# Autodesk Inventor assembly: Subensamble_mesa
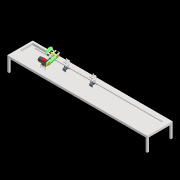
[picture p0: Inventor's stored thumbnail of the model, 180x180]
Saved by Autodesk Inventor 2021 (Build 250183000, 183)
## iProperties
Created: 2021-04-29
Part Number: Subensamble_mesa
Document SubType Name: Assembly
Designer: Admin
Author: Admin
## Documents named in this file (18)
- C:\Users\maaro\Documents\UNAL\Automatización de Procesos de Manufactura\Github\Proyecto_APM\CADs estaciones a automatizar\Estación corte\Subensamble_mesa.iam
- C:\Users\maaro\Documents\UNAL\Automatización de Procesos de Manufactura\Github\Proyecto_APM\CADs estaciones a automatizar\Estación corte\Mesa_cortadora.ipt
- C:\Users\maaro\Documents\UNAL\Automatización de Procesos de Manufactura\Github\Proyecto_APM\CADs estaciones a automatizar\Estación corte\Pata_mesa.ipt
- C:\Users\maaro\Documents\UNAL\Automatización de Procesos de Manufactura\Github\Proyecto_APM\CADs estaciones a automatizar\Estación corte\Subensamble_cortadora.iam
- C:\Users\maaro\Documents\UNAL\Automatización de Procesos de Manufactura\Github\Proyecto_APM\CADs estaciones a automatizar\Estación corte\Tubo-2_1_8.ipt
- C:\Users\maaro\Documents\UNAL\Automatización de Procesos de Manufactura\Github\Proyecto_APM\CADs estaciones a automatizar\Estación corte\Base soporte tubos.ipt
- C:\Users\maaro\Documents\UNAL\Automatización de Procesos de Manufactura\Github\Proyecto_APM\CADs estaciones a automatizar\Estación corte\193992 DSNU-32-60-PPS-A---(60PPSA---00--0-------0).iam
- C:\Users\maaro\Documents\UNAL\Automatización de Procesos de Manufactura\Github\Proyecto_APM\CADs estaciones a automatizar\Estación corte\Eje roscado base soporte tubo.ipt
- C:\Users\maaro\Documents\UNAL\Automatización de Procesos de Manufactura\Github\Proyecto_APM\CADs estaciones a automatizar\Estación corte\Soporte Superior Tubos.ipt
- C:\Users\maaro\Documents\UNAL\Automatización de Procesos de Manufactura\Github\Proyecto_APM\CADs estaciones a automatizar\Estación corte\Soporte Pistón.ipt
- C:\Users\maaro\Documents\Inventor\Content Center Files\R2021\en-US\ISO 4035(2)\ISO 4035 - M16 - ISO.ipt
- C:\Users\maaro\Documents\UNAL\Automatización de Procesos de Manufactura\Github\Proyecto_APM\CADs estaciones a automatizar\Estación corte\Eje roscado base soporte tubo_MIR.ipt
- C:\Users\maaro\Documents\UNAL\Automatización de Procesos de Manufactura\Github\Proyecto_APM\CADs estaciones a automatizar\Estación corte\193992 DSNU-32-60-PPS-A---(60PPSA---00--0-------0)_MIR.iam
- C:\Users\maaro\Documents\UNAL\Automatización de Procesos de Manufactura\Github\Proyecto_APM\CADs estaciones a automatizar\Estación corte\Base soporte tubos_MIR.ipt
- C:\Users\maaro\Documents\UNAL\Automatización de Procesos de Manufactura\Github\Proyecto_APM\CADs estaciones a automatizar\Estación corte\Eje roscado base soporte tubo_MIR1.ipt
- C:\Users\maaro\Documents\UNAL\Automatización de Procesos de Manufactura\Github\Proyecto_APM\CADs estaciones a automatizar\Estación corte\Soporte Superior Tubos_MIR.ipt
- C:\Users\maaro\Documents\UNAL\Automatización de Procesos de Manufactura\Github\Proyecto_APM\CADs estaciones a automatizar\Estación corte\Soporte Pistón_MIR.ipt
- C:\Users\maaro\Documents\UNAL\Automatización de Procesos de Manufactura\Github\Proyecto_APM\CADs estaciones a automatizar\Estación corte\Eje roscado base soporte tubo_MIR_MIR.ipt
## Components (36 placed, 17 different names)
1. Mesa_cortadora:1 — Coincidencia:1, Coincidencia:2, Coincidencia:3, Coincidencia:4, Coincidencia:5, Coincidencia:6, Coincidencia:7, Coincidencia:8, Coincidencia:9, Coincidencia:10, Coincidencia:11, Coincidencia:12, Coincidencia:13, Coincidencia:14, Mate:15, Flush:1, Flush:2, Mate:16, Flush:3, Mate:80, Flush:17
2. Pata_mesa:1 — Coincidencia:7, Coincidencia:8, Coincidencia:9
3. Pata_mesa:2 — Coincidencia:1, Coincidencia:2, Coincidencia:3
4. Pata_mesa:3 — Coincidencia:4, Coincidencia:5, Coincidencia:6
5. Pata_mesa:4 — Coincidencia:10, Coincidencia:11, Coincidencia:12
6. Subensamble_cortadora:1 [sub-assembly] — Coincidencia:13, Coincidencia:14
7. Tubo-2_1_8:1 — Tangent:1, Tangent:2, Flush:7
8. Base soporte tubos:1 — Mate:15, Tangent:1, Tangent:2, Flush:1, Flush:2
9. 193992 DSNU-32-60-PPS-A---(60PPSA---00--0-------0):2 [sub-assembly] — Mate:18, Flush:10, Flush:11
10. Base soporte tubos:2 — Mate:16, Flush:3, Flush:5, Flush:6, Flush:8, Flush:9, Mate:23, Mate:25, Mate:31, Mate:36, Mate:37, Mate:38, Flush:12
11. Eje roscado base soporte tubo:1 — Flush:5, Flush:6, Mate:20, Mate:22, Mate:24, Mate:26, Mate:31, Mate:32, Mate:33
12. Soporte Superior Tubos:1 — Flush:7, Flush:8, Flush:9, Mate:18, Symmetry:1, Mate:33
13. Soporte Pistón:1 — Flush:10, Flush:11, Mate:19, Mate:21, Symmetry:1, Mate:32, Mate:34, Mate:35, Flush:13, Mate:39
14. ISO 4035 M16:1 — Mate:21, Mate:22
15. ISO 4035 M16:2 — Mate:19, Mate:20
16. ISO 4035 M16:3 — Mate:23, Mate:24
17. ISO 4035 M16:4 — Mate:25, Mate:26
18. Eje roscado base soporte tubo_MIR:1 — Mate:27, Mate:28, Mate:29, Mate:30, Mate:38, Flush:12, Flush:13, Mate:39
19. ISO 4035 M16:5 — Mate:27, Mate:34
20. ISO 4035 M16:6 — Mate:28, Mate:35
21. ISO 4035 M16:7 — Mate:29, Mate:37
22. ISO 4035 M16:8 — Mate:30, Mate:36
23. 193992 DSNU-32-60-PPS-A---(60PPSA---00--0-------0)_MIR:1 [sub-assembly] — Mate:44, Mate:48, Mate:49
24. Base soporte tubos_MIR:1 — Mate:40, Mate:41, Mate:42, Mate:45, Mate:46, Mate:55, Mate:57, Flush:16, Mate:59, Mate:64, Mate:66, Mate:72, Mate:74, Mate:76, Mate:78, Mate:80, Flush:17
25. Eje roscado base soporte tubo_MIR1:1 — Mate:40, Mate:41, Mate:42, Mate:43, Mate:47, Mate:50, Mate:52, Mate:73, Mate:77
26. Soporte Superior Tubos_MIR:1 — Mate:43, Mate:44, Mate:45, Mate:46, Symmetry:2
27. Soporte Pistón_MIR:1 — Mate:47, Mate:48, Mate:49, Symmetry:2, Mate:58, Flush:15, Mate:62, Mate:69, Mate:71, Mate:81, Mate:82
28. ISO 4035 M16:9 — Mate:50, Mate:82
29. ISO 4035 M16:10 — Mate:52, Mate:71
30. ISO 4035 M16:11 — Mate:55, Mate:76, Mate:77
31. ISO 4035 M16:12 — Mate:57, Mate:72, Mate:73
32. Eje roscado base soporte tubo_MIR_MIR:1 — Mate:58, Flush:15, Flush:16, Mate:59, Mate:61, Mate:70, Mate:75, Mate:79
33. ISO 4035 M16:13 — Mate:61, Mate:81
34. ISO 4035 M16:14 — Mate:62, Mate:69, Mate:70
35. ISO 4035 M16:15 — Mate:64, Mate:78, Mate:79
36. ISO 4035 M16:16 — Mate:66, Mate:74, Mate:75
## Relationships (91: Mate 72, Flush 15, Tangent 2, Symmetry 2)
- Coincidencia:1 [Mate]: Mesa_cortadora:1 ↔ Pata_mesa:2
- Coincidencia:2 [Mate]: Mesa_cortadora:1 ↔ Pata_mesa:2
- Coincidencia:3 [Mate]: Mesa_cortadora:1 ↔ Pata_mesa:2
- Coincidencia:4 [Mate]: Mesa_cortadora:1 ↔ Pata_mesa:3
- Coincidencia:5 [Mate]: Mesa_cortadora:1 ↔ Pata_mesa:3
- Coincidencia:6 [Mate]: Mesa_cortadora:1 ↔ Pata_mesa:3
- Coincidencia:7 [Mate]: Mesa_cortadora:1 ↔ Pata_mesa:1
- Coincidencia:8 [Mate]: Mesa_cortadora:1 ↔ Pata_mesa:1
- Coincidencia:9 [Mate]: Mesa_cortadora:1 ↔ Pata_mesa:1
- Coincidencia:10 [Mate]: Mesa_cortadora:1 ↔ Pata_mesa:4
- Coincidencia:11 [Mate]: Mesa_cortadora:1 ↔ Pata_mesa:4
- Coincidencia:12 [Mate]: Mesa_cortadora:1 ↔ Pata_mesa:4
- Coincidencia:13 [Mate]: Mesa_cortadora:1 ↔ Subensamble_cortadora:1
- Coincidencia:14 [Mate]: Mesa_cortadora:1 ↔ Subensamble_cortadora:1
- Mate:15: Mesa_cortadora:1 ↔ Base soporte tubos:1
- Tangent:1: Tubo-2_1_8:1 ↔ Base soporte tubos:1
- Tangent:2: Tubo-2_1_8:1 ↔ Base soporte tubos:1
- Flush:1 (297.3 mm): Mesa_cortadora:1 ↔ Base soporte tubos:1
- Flush:2 (1220 mm): Mesa_cortadora:1 ↔ Base soporte tubos:1
- Mate:16: Mesa_cortadora:1 ↔ Base soporte tubos:2
- Flush:3 (297 mm): Mesa_cortadora:1 ↔ Base soporte tubos:2
- Flush:5: Base soporte tubos:2 ↔ Eje roscado base soporte tubo:1
- Flush:6 (20 mm): Base soporte tubos:2 ↔ Eje roscado base soporte tubo:1
- Flush:7: Tubo-2_1_8:1 ↔ Soporte Superior Tubos:1
- Flush:8: Base soporte tubos:2 ↔ Soporte Superior Tubos:1
- Flush:9: Base soporte tubos:2 ↔ Soporte Superior Tubos:1
- Mate:18: 193992 DSNU-32-60-PPS-A---(60PPSA---00--0-------0):2 ↔ Soporte Superior Tubos:1
- Flush:10: 193992 DSNU-32-60-PPS-A---(60PPSA---00--0-------0):2 ↔ Soporte Pistón:1
- Flush:11: 193992 DSNU-32-60-PPS-A---(60PPSA---00--0-------0):2 ↔ Soporte Pistón:1
- Mate:19: Soporte Pistón:1 ↔ ISO 4035 M16:2
- Mate:20: Eje roscado base soporte tubo:1 ↔ ISO 4035 M16:2
- Mate:21: Soporte Pistón:1 ↔ ISO 4035 M16:1
- Mate:22: Eje roscado base soporte tubo:1 ↔ ISO 4035 M16:1
- Mate:23: Base soporte tubos:2 ↔ ISO 4035 M16:3
- Mate:24: Eje roscado base soporte tubo:1 ↔ ISO 4035 M16:3
- Mate:25: Base soporte tubos:2 ↔ ISO 4035 M16:4
- Mate:26: Eje roscado base soporte tubo:1 ↔ ISO 4035 M16:4
- Symmetry:1: Soporte Superior Tubos:1 ↔ Soporte Pistón:1
- Mate:27: Eje roscado base soporte tubo_MIR:1 ↔ ISO 4035 M16:5
- Mate:28: Eje roscado base soporte tubo_MIR:1 ↔ ISO 4035 M16:6
- Mate:29: Eje roscado base soporte tubo_MIR:1 ↔ ISO 4035 M16:7
- Mate:30: Eje roscado base soporte tubo_MIR:1 ↔ ISO 4035 M16:8
- Mate:31: Base soporte tubos:2 ↔ Eje roscado base soporte tubo:1
- Mate:32: Eje roscado base soporte tubo:1 ↔ Soporte Pistón:1
- Mate:33: Eje roscado base soporte tubo:1 ↔ Soporte Superior Tubos:1
- Mate:34: Soporte Pistón:1 ↔ ISO 4035 M16:5
- Mate:35: Soporte Pistón:1 ↔ ISO 4035 M16:6
- Mate:36: Base soporte tubos:2 ↔ ISO 4035 M16:8
- Mate:37: Base soporte tubos:2 ↔ ISO 4035 M16:7
- Mate:38: Base soporte tubos:2 ↔ Eje roscado base soporte tubo_MIR:1
- Flush:12 (-20 mm): Base soporte tubos:2 ↔ Eje roscado base soporte tubo_MIR:1
- Flush:13 (-27.5 mm): Soporte Pistón:1 ↔ Eje roscado base soporte tubo_MIR:1
- Mate:39: Soporte Pistón:1 ↔ Eje roscado base soporte tubo_MIR:1
- Mate:40: Base soporte tubos_MIR:1 ↔ Eje roscado base soporte tubo_MIR1:1
- Mate:41 (20 mm): Base soporte tubos_MIR:1 ↔ Eje roscado base soporte tubo_MIR1:1
- Mate:42: Base soporte tubos_MIR:1 ↔ Eje roscado base soporte tubo_MIR1:1
- Mate:43: Eje roscado base soporte tubo_MIR1:1 ↔ Soporte Superior Tubos_MIR:1
- Mate:44: 193992 DSNU-32-60-PPS-A---(60PPSA---00--0-------0)_MIR:1 ↔ Soporte Superior Tubos_MIR:1
- Mate:45: Base soporte tubos_MIR:1 ↔ Soporte Superior Tubos_MIR:1
- Mate:46: Base soporte tubos_MIR:1 ↔ Soporte Superior Tubos_MIR:1
- Mate:47: Eje roscado base soporte tubo_MIR1:1 ↔ Soporte Pistón_MIR:1
- Mate:48: 193992 DSNU-32-60-PPS-A---(60PPSA---00--0-------0)_MIR:1 ↔ Soporte Pistón_MIR:1
- Mate:49: 193992 DSNU-32-60-PPS-A---(60PPSA---00--0-------0)_MIR:1 ↔ Soporte Pistón_MIR:1
- Mate:50: Eje roscado base soporte tubo_MIR1:1 ↔ ISO 4035 M16:9
- Mate:52: Eje roscado base soporte tubo_MIR1:1 ↔ ISO 4035 M16:10
- Mate:55: Base soporte tubos_MIR:1 ↔ ISO 4035 M16:11
- Mate:57: Base soporte tubos_MIR:1 ↔ ISO 4035 M16:12
- Symmetry:2: Soporte Superior Tubos_MIR:1 ↔ Soporte Pistón_MIR:1
- Mate:58: Soporte Pistón_MIR:1 ↔ Eje roscado base soporte tubo_MIR_MIR:1
- Flush:15 (-27.5 mm): Soporte Pistón_MIR:1 ↔ Eje roscado base soporte tubo_MIR_MIR:1
- Flush:16 (-20 mm): Base soporte tubos_MIR:1 ↔ Eje roscado base soporte tubo_MIR_MIR:1
- Mate:59: Base soporte tubos_MIR:1 ↔ Eje roscado base soporte tubo_MIR_MIR:1
- Mate:61: Eje roscado base soporte tubo_MIR_MIR:1 ↔ ISO 4035 M16:13
- Mate:62: Soporte Pistón_MIR:1 ↔ ISO 4035 M16:14
- Mate:64: Base soporte tubos_MIR:1 ↔ ISO 4035 M16:15
- Mate:66: Base soporte tubos_MIR:1 ↔ ISO 4035 M16:16
- Mate:69: Soporte Pistón_MIR:1 ↔ ISO 4035 M16:14
- Mate:70: Eje roscado base soporte tubo_MIR_MIR:1 ↔ ISO 4035 M16:14
- Mate:71: Soporte Pistón_MIR:1 ↔ ISO 4035 M16:10
- Mate:72: Base soporte tubos_MIR:1 ↔ ISO 4035 M16:12
- Mate:73: Eje roscado base soporte tubo_MIR1:1 ↔ ISO 4035 M16:12
- Mate:74: Base soporte tubos_MIR:1 ↔ ISO 4035 M16:16
- Mate:75: Eje roscado base soporte tubo_MIR_MIR:1 ↔ ISO 4035 M16:16
- Mate:76: Base soporte tubos_MIR:1 ↔ ISO 4035 M16:11
- Mate:77: Eje roscado base soporte tubo_MIR1:1 ↔ ISO 4035 M16:11
- Mate:78: Base soporte tubos_MIR:1 ↔ ISO 4035 M16:15
- Mate:79: Eje roscado base soporte tubo_MIR_MIR:1 ↔ ISO 4035 M16:15
- Mate:80: Mesa_cortadora:1 ↔ Base soporte tubos_MIR:1
- Mate:81: Soporte Pistón_MIR:1 ↔ ISO 4035 M16:13
- Mate:82: Soporte Pistón_MIR:1 ↔ ISO 4035 M16:9
- Flush:17 (297 mm): Mesa_cortadora:1 ↔ Base soporte tubos_MIR:1
